# Autodesk Inventor assembly: assembly_arm_2
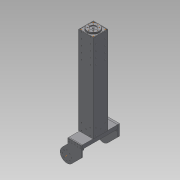
[picture p0: Inventor's stored thumbnail of the model, 180x180]
Saved by Autodesk Inventor 2017 (Build 210142000, 142)
## iProperties
Part Number: assembly_arm_2
Material: Generisch
Document SubType Name: Assembly
Designer: Max
Author: Max
## Documents named in this file (5)
- C:\Users\Max\Desktop\SENAI\robot_arm_new\assembly_arm_2.iam
- C:\Users\Max\Desktop\SENAI\robot_arm_new\complex_frame\pro_complex_frame_assembly.iam
- C:\Users\Max\Desktop\SENAI\robot_arm_new\cube_square_tube.ipt
- C:\Users\Max\Desktop\SENAI\robot_arm_new\h54-200-s500-r.ipt
- C:\Users\Max\Desktop\SENAI\robot_arm_new\complex_frame\square_tube_2.ipt
## Components (4 placed, 4 different names)
1. pro_complex_frame_assembly:1 [sub-assembly] — Passend:1, Passend:2, Passend:3, Winkel:1, Passend:10, Passend:11, Passend:12
2. cube_square_tube:1 — Passend:1, Passend:2, Passend:3, Passend:4, Passend:5, Passend:6
3. h54-200-s500-r:1 — Passend:7, Passend:8
4. square_tube_2:1 — Passend:4, Passend:5, Passend:6, Passend:7, Passend:8
## Relationships (12: Mate 11, Angle 1)
- Passend:1 [Mate]: pro_complex_frame_assembly:1 ↔ cube_square_tube:1
- Passend:2 [Mate]: pro_complex_frame_assembly:1 ↔ cube_square_tube:1
- Passend:3 [Mate]: pro_complex_frame_assembly:1 ↔ cube_square_tube:1
- Passend:4 [Mate]: cube_square_tube:1 ↔ square_tube_2:1
- Passend:5 [Mate]: cube_square_tube:1 ↔ square_tube_2:1
- Passend:6 [Mate]: cube_square_tube:1 ↔ square_tube_2:1
- Passend:7 [Mate]: h54-200-s500-r:1 ↔ square_tube_2:1
- Passend:8 [Mate]: h54-200-s500-r:1 ↔ square_tube_2:1
- Winkel:1 [Angle] (0 deg): pro_complex_frame_assembly:1
- Passend:10 [Mate] (69 mm): pro_complex_frame_assembly:1
- Passend:11 [Mate]: pro_complex_frame_assembly:1
- Passend:12 [Mate]: pro_complex_frame_assembly:1
